# Autodesk Inventor assembly: Gantry Table With Chucks
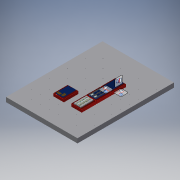
[picture p0: Inventor's stored thumbnail of the model, 180x180]
Saved by Autodesk Inventor 2019.4 (Build 234330000, 330)
## iProperties
Created: 2021-01-12
Part Number: Gantry Table With Chucks
Document SubType Name: Assembly
Designer: caleb
Author: caleb
## Documents named in this file (6)
- C:\Users\cfang\Desktop\nebraska-silicon-lab\CAD\ETL\Module Assembly\Gantry Table With Chucks.iam
- C:\Users\cfang\Desktop\nebraska-silicon-lab\CAD\ETL\Module Assembly\Gantry Base.ipt
- C:\Users\cfang\Desktop\nebraska-silicon-lab\CAD\ETL\Module Assembly\Chuck with Assembly Plate.iam
- C:\Users\cfang\Desktop\nebraska-silicon-lab\CAD\ETL\Module Assembly\Chuck with BBM Staging Plate.iam
- C:\Users\cfang\Desktop\nebraska-silicon-lab\CAD\ETL\Module Assembly\Chuck with Glue Reservoir Plate.iam
- C:\Users\cfang\Desktop\nebraska-silicon-lab\CAD\ETL\Module Assembly\Chuck with Glue Stamp Staging Plate.iam
## Components (5 placed, 5 different names)
1. Gantry Base:1 — Mate:1, Mate:2, Mate:3, Mate:4, Angle:1, Angle:2, Angle:3, Angle:4, Insert:3, Insert:4, Insert:5, Insert:6
2. Chuck with Assembly Plate:1 [sub-assembly] — Mate:1, Angle:1, Insert:4
3. Chuck with BBM Staging Plate:1 [sub-assembly] — Mate:2, Angle:2, Insert:3
4. Chuck with Glue Reservoir Plate:1 [sub-assembly] — Mate:3, Angle:3, Insert:5
5. Chuck with Glue Stamp Staging Plate:1 [sub-assembly] — Mate:4, Angle:4, Insert:6
## Relationships (12: Mate 4, Angle 4, Insert 4)
- Mate:1: Gantry Base:1 ↔ Chuck with Assembly Plate:1
- Mate:2: Gantry Base:1 ↔ Chuck with BBM Staging Plate:1
- Mate:3: Gantry Base:1 ↔ Chuck with Glue Reservoir Plate:1
- Mate:4: Gantry Base:1 ↔ Chuck with Glue Stamp Staging Plate:1
- Angle:1 (0 deg): Gantry Base:1 ↔ Chuck with Assembly Plate:1
- Angle:2 (0 deg): Gantry Base:1 ↔ Chuck with BBM Staging Plate:1
- Angle:3 (0 deg): Gantry Base:1 ↔ Chuck with Glue Reservoir Plate:1
- Angle:4 (0 deg): Gantry Base:1 ↔ Chuck with Glue Stamp Staging Plate:1
- Insert:3: Gantry Base:1 ↔ Chuck with BBM Staging Plate:1
- Insert:4: Gantry Base:1 ↔ Chuck with Assembly Plate:1
- Insert:5: Gantry Base:1 ↔ Chuck with Glue Reservoir Plate:1
- Insert:6: Gantry Base:1 ↔ Chuck with Glue Stamp Staging Plate:1
